# Autodesk Inventor assembly: Simulation_module_2
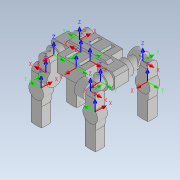
[picture p0: Inventor's stored thumbnail of the model, 180x180]
Saved by Autodesk Inventor 2020 (Build 240168000, 168)
## iProperties
Created: 2021-01-12
Part Number: Simulation_module_2
Document SubType Name: Assembly
Designer: DELL
Author: DELL
## Documents named in this file (9)
- F:\SoftRobot2.0\FlexipodHardware2.0\FlexipodHardware\Flexipod2.0\Cadquery_module\v7.0\Simulation_module.iam
- F:\SoftRobot2.0\FlexipodHardware2.0\FlexipodHardware\Flexipod2.0\Cadquery_module\v7.0\body.ipt
- F:\SoftRobot2.0\FlexipodHardware2.0\FlexipodHardware\Flexipod2.0\Cadquery_module\v7.0\hip.ipt
- F:\SoftRobot2.0\FlexipodHardware2.0\FlexipodHardware\Flexipod2.0\Cadquery_module\v7.0\thigh.ipt
- F:\SoftRobot2.0\FlexipodHardware2.0\FlexipodHardware\Flexipod2.0\Cadquery_module\v7.0\shank.ipt
- F:\SoftRobot2.0\FlexipodHardware2.0\FlexipodHardware\Flexipod2.0\Cadquery_module\v7.0\hip_back.ipt
- F:\SoftRobot2.0\FlexipodHardware2.0\FlexipodHardware\Flexipod2.0\Cadquery_module\v7.0\hip_back_mirror.ipt
- F:\SoftRobot2.0\FlexipodHardware2.0\FlexipodHardware\Flexipod2.0\Cadquery_module\v7.0\hip_mirror.ipt
- F:\SoftRobot2.0\FlexipodHardware2.0\FlexipodHardware\Flexipod2.0\robot_2021_1_27\robot.iam
## Components (14 placed, 8 different names)
1. body:1 — Flush:1, Flush:2, Flush:3, Angle:2, Mate:7, Mate:8, Angle:4, Angle:5, Mate:13, Mate:14, Angle:7, Mate:27, Mate:28, Angle:15, Mate:33, Mate:34, Angle:16
2. hip:1 — Mate:7, Mate:8, Angle:4, Mate:10, Mate:32
3. thigh:11 — Angle:2, Mate:6, Flush:4, Mate:25, Angle:12, Mate:35, Mate:36, Angle:16
4. thigh:12 — Mate:10, Angle:5, Mate:12, Flush:8, Angle:11, Mate:32
5. shank:7 — Mate:12, Flush:8, Angle:11
6. shank:8 — Mate:6, Flush:5, Mate:25, Angle:12
7. hip_back:1 — Mate:13, Mate:14, Angle:7, Mate:18, Angle:9, Flush:7, Mate:31
8. thigh:13 — Mate:18, Angle:9, Mate:24, Flush:9, Angle:14, Mate:31
9. thigh:14 — Mate:22, Mate:26, Angle:13, Mate:29, Mate:30, Angle:17
10. shank:9 — Mate:22, Mate:26, Angle:13
11. shank:10 — Mate:24, Flush:6, Flush:9, Angle:14
12. hip_back_mirror:1 — Mate:27, Mate:28, Angle:15, Mate:29, Mate:30, Angle:17
13. hip_mirror:1 — Mate:33, Mate:34, Mate:35, Mate:36
14. robot:1 [sub-assembly]
## Relationships (43: Mate 22, Angle 12, Flush 9)
- Flush:1: body:1
- Flush:2: body:1
- Flush:3: body:1
- Angle:2 (0 deg): body:1 ↔ thigh:11
- Mate:6: thigh:11 ↔ shank:8
- Mate:7: body:1 ↔ hip:1
- Mate:8: body:1 ↔ hip:1
- Angle:4 (0 deg): body:1 ↔ hip:1
- Mate:10: hip:1 ↔ thigh:12
- Angle:5 (0 deg): body:1 ↔ thigh:12
- Mate:12: thigh:12 ↔ shank:7
- Mate:13: body:1 ↔ hip_back:1
- Mate:14: body:1 ↔ hip_back:1
- Angle:7 (0 deg): body:1 ↔ hip_back:1
- Mate:18: hip_back:1 ↔ thigh:13
- Angle:9 (0 deg): hip_back:1 ↔ thigh:13
- Mate:22: thigh:14 ↔ shank:9
- Mate:24: thigh:13 ↔ shank:10
- Flush:4: thigh:11
- Flush:5: shank:8
- Flush:6: shank:10
- Flush:7: hip_back:1
- Flush:8: thigh:12 ↔ shank:7
- Mate:25: thigh:11 ↔ shank:8
- Flush:9: thigh:13 ↔ shank:10
- Mate:26: thigh:14 ↔ shank:9
- Angle:11 (180 deg): thigh:12 ↔ shank:7
- Angle:12 (0 deg): thigh:11 ↔ shank:8
- Angle:13 (0 deg): thigh:14 ↔ shank:9
- Angle:14 (180 deg): thigh:13 ↔ shank:10
- Mate:27: body:1 ↔ hip_back_mirror:1
- Mate:28: body:1 ↔ hip_back_mirror:1
- Angle:15 (0 deg): body:1 ↔ hip_back_mirror:1
- Mate:29: thigh:14 ↔ hip_back_mirror:1
- Mate:30: thigh:14 ↔ hip_back_mirror:1
- Mate:31: hip_back:1 ↔ thigh:13
- Mate:32: hip:1 ↔ thigh:12
- Mate:33: body:1 ↔ hip_mirror:1
- Mate:34: body:1 ↔ hip_mirror:1
- Mate:35: thigh:11 ↔ hip_mirror:1
- Mate:36: thigh:11 ↔ hip_mirror:1
- Angle:16 (0 deg): body:1 ↔ thigh:11
- Angle:17 (0 deg): thigh:14 ↔ hip_back_mirror:1
